# Autodesk Inventor assembly: DriveTrainMotor+Mount
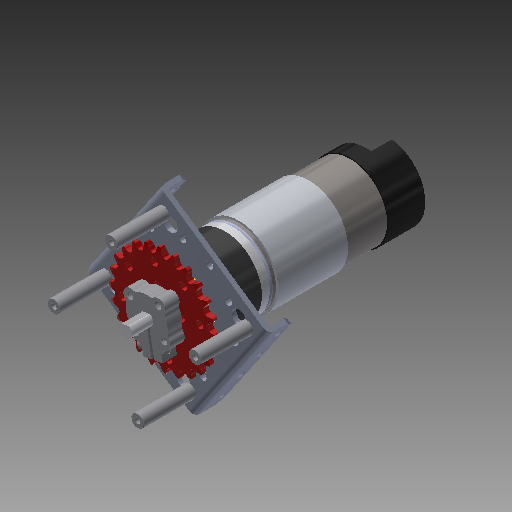
[picture p0: Inventor's stored thumbnail of the model, 512x512]
Saved by Autodesk Inventor 2018 (Build 220112000, 112)
## iProperties
Created: 2017-11-14
Part Number: DriveTrainMotor+Mount
Document SubType Name: Assembly
Designer: ball
Author: ball
## Documents named in this file (7)
- C:\FTC\2017Robot\DriveTrainMotor+Mount.iam
- C:\FTC\Andymark\am-3461a+NeveRest+Orbital+3.7+REV2.ipt
- C:\FTC\Andymark\am-3474 actobotics hole pattern.ipt
- C:\FTC\Actobotics\615 parts\615106.ipt
- C:\FTC\Actobotics\545 parts\545618 assembly.ipt
- C:\FTC\StepLibraries\Screws\M3x6 SHCS.ipt
- C:\FTC\Actobotics\633 parts\633130.ipt
## Components (12 placed, 6 different names)
1. am-3461a+NeveRest+Orbital+3.7+REV2:1 — Mate:1, Mate:2, Mate:3, Mate:4, Mate:16, Mate:17, Flush:1
2. am-3474 actobotics hole pattern:2 — Mate:1, Mate:2, Mate:3, Mate:4, Mate:5, Mate:6, Mate:7, Mate:8, Mate:9, Mate:10, Mate:11, Mate:12, Mate:18, Mate:19, Mate:20, Mate:21, Mate:22, Mate:23, Mate:24, Mate:25
3. 615106:1 — Mate:13, Mate:14, Mate:15, Mate:16
4. 545618 assembly:1 — Mate:13, Mate:14, Mate:15, Mate:17, Flush:1
5. M3x6 SHCS:1 — Mate:7, Mate:10
6. M3x6 SHCS:2 — Mate:8, Mate:12
7. M3x6 SHCS:3 — Mate:6, Mate:11
8. M3x6 SHCS:4 — Mate:5, Mate:9
9. 633130:1 — Mate:18, Mate:22
10. 633130:2 — Mate:19, Mate:23
11. 633130:3 — Mate:20, Mate:24
12. 633130:4 — Mate:21, Mate:25
## Relationships (26: Mate 25, Flush 1)
- Mate:1: am-3461a+NeveRest+Orbital+3.7+REV2:1 ↔ am-3474 actobotics hole pattern:2
- Mate:2: am-3461a+NeveRest+Orbital+3.7+REV2:1 ↔ am-3474 actobotics hole pattern:2
- Mate:3: am-3461a+NeveRest+Orbital+3.7+REV2:1 ↔ am-3474 actobotics hole pattern:2
- Mate:4: am-3461a+NeveRest+Orbital+3.7+REV2:1 ↔ am-3474 actobotics hole pattern:2
- Mate:5: am-3474 actobotics hole pattern:2 ↔ M3x6 SHCS:4
- Mate:6: am-3474 actobotics hole pattern:2 ↔ M3x6 SHCS:3
- Mate:7: am-3474 actobotics hole pattern:2 ↔ M3x6 SHCS:1
- Mate:8: am-3474 actobotics hole pattern:2 ↔ M3x6 SHCS:2
- Mate:9: am-3474 actobotics hole pattern:2 ↔ M3x6 SHCS:4
- Mate:10: am-3474 actobotics hole pattern:2 ↔ M3x6 SHCS:1
- Mate:11: am-3474 actobotics hole pattern:2 ↔ M3x6 SHCS:3
- Mate:12: am-3474 actobotics hole pattern:2 ↔ M3x6 SHCS:2
- Mate:13: 615106:1 ↔ 545618 assembly:1
- Mate:14: 615106:1 ↔ 545618 assembly:1
- Mate:15: 615106:1 ↔ 545618 assembly:1
- Mate:16: am-3461a+NeveRest+Orbital+3.7+REV2:1 ↔ 615106:1
- Mate:17: am-3461a+NeveRest+Orbital+3.7+REV2:1 ↔ 545618 assembly:1
- Flush:1 (-10.16 mm): am-3461a+NeveRest+Orbital+3.7+REV2:1 ↔ 545618 assembly:1
- Mate:18: am-3474 actobotics hole pattern:2 ↔ 633130:1
- Mate:19: am-3474 actobotics hole pattern:2 ↔ 633130:2
- Mate:20: am-3474 actobotics hole pattern:2 ↔ 633130:3
- Mate:21: am-3474 actobotics hole pattern:2 ↔ 633130:4
- Mate:22: am-3474 actobotics hole pattern:2 ↔ 633130:1
- Mate:23: am-3474 actobotics hole pattern:2 ↔ 633130:2
- Mate:24: am-3474 actobotics hole pattern:2 ↔ 633130:3
- Mate:25: am-3474 actobotics hole pattern:2 ↔ 633130:4
